# Autodesk Inventor assembly: МД.001.1000 - Захват
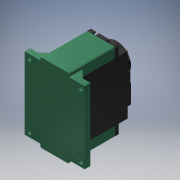
[picture p0: Inventor's stored thumbnail of the model, 180x180]
Saved by Autodesk Inventor 2019 (Build 230136000, 136)
## iProperties
Created: 2019-12-30
Part Number: МД.001.1000 - Захват
Material: Типовые
Document SubType Name: Assembly
Designer: Петров Иван
Author: Петров Иван
## Documents named in this file (3)
- E:\IVAN\Ivan_desktop\GitHub\Arm_manip\hardware\МД.001.1000 - Захват.iam
- E:\IVAN\Ivan_desktop\GitHub\Arm_manip\hardware\МД.001.1001 - Опора захвата.ipt
- E:\IVAN\Ivan_desktop\GitHub\Arm_manip\hardware\Standart_things\tower prone.ipt
## Components (2 placed, 2 different names)
1. МД.001.1001 - Опора захвата:1 — Совмещение:1, Совмещение:2, Совмещение:3
2. tower prone:1 — Совмещение:1, Совмещение:2, Совмещение:3
## Relationships (3: Mate 3)
- Совмещение:1 [Mate]: МД.001.1001 - Опора захвата:1 ↔ tower prone:1
- Совмещение:2 [Mate]: МД.001.1001 - Опора захвата:1 ↔ tower prone:1
- Совмещение:3 [Mate]: МД.001.1001 - Опора захвата:1 ↔ tower prone:1
